# Autodesk Inventor assembly: bunny bot 2013 idea 2.2
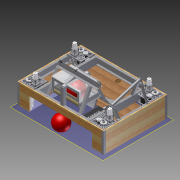
[picture p0: Inventor's stored thumbnail of the model, 180x180]
Saved by Autodesk Inventor 2012 (Build 160160000, 160)
## iProperties
Created: 2013-09-01
Part Number: bunny bot 2013 idea 2.2
Document SubType Name: Assembly
Designer: Bryce
Author: Bryce
## Documents named in this file (30)
- C:\Users\Bryce\Dropbox\Inventor Design Project Files\Independent Swerves\Inventor 2012\bunny bot 2013 idea 2.2.iam
- C:\Users\Bryce\Dropbox\Inventor Design Project Files\Independent Swerves\Inventor 2012\FULL SWERVE DRIVE ASSEMBLY!  2!.iam
- C:\Users\Bryce\Dropbox\Inventor Design Project Files\Independent Swerves\Inventor 2012\frame U 1 by 3.ipt
- C:\Users\Bryce\Dropbox\Inventor Design Project Files\Independent Swerves\Inventor 2012\frame U 1 by 3 long.ipt
- C:\Users\Bryce\Dropbox\Inventor Design Project Files\Independent Swerves\Inventor 2012\plywood side pannel.ipt
- C:\Users\Bryce\Dropbox\Inventor Design Project Files\Independent Swerves\Inventor 2012\plywood back pannel 2.ipt
- C:\Users\Bryce\Dropbox\Inventor Design Project Files\Independent Swerves\Inventor 2012\dozer side pannel.ipt
- C:\Users\Bryce\Dropbox\Inventor Design Project Files\Independent Swerves\Inventor 2012\plywood front pannel 2.ipt
- C:\Users\Bryce\Dropbox\Inventor Design Project Files\Independent Swerves\Inventor 2012\dodge ball.ipt
- C:\Users\Bryce\Dropbox\Inventor Design Project Files\Independent Swerves\Inventor 2012\dozer side end mount.ipt
- C:\Users\Bryce\Dropbox\Inventor Design Project Files\Independent Swerves\Inventor 2012\bumper corner bracket.ipt
- C:\Users\Bryce\Dropbox\Inventor Design Project Files\Independent Swerves\Inventor 2012\dozer side mid mount.ipt
- C:\Users\Bryce\Dropbox\Inventor Design Project Files\Independent Swerves\Inventor 2012\frame box 1 by 3.ipt
- C:\Users\Bryce\Dropbox\Inventor Design Project Files\Independent Swerves\Inventor 2012\belly pan.ipt
- C:\Users\Bryce\Dropbox\Inventor Design Project Files\Independent Swerves\Inventor 2012\8 ball frame tube.ipt
- C:\Users\Bryce\Dropbox\Inventor Design Project Files\Independent Swerves\Inventor 2012\manipulator pnumaitic pivot.ipt
- C:\Users\Bryce\Dropbox\Inventor Design Project Files\Independent Swerves\Inventor 2012\bunny throw base 1.ipt
- C:\Users\Bryce\Dropbox\Inventor Design Project Files\Independent Swerves\Inventor 2012\bunny throw base 2.ipt
- C:\Users\Bryce\Dropbox\Inventor Design Project Files\Independent Swerves\Inventor 2012\1' by 1'' dia piston.ipt
- C:\Users\Bryce\Dropbox\Inventor Design Project Files\Independent Swerves\Inventor 2012\bunny throw piston bracket.ipt
- C:\Users\Bryce\Dropbox\Inventor Design Project Files\Independent Swerves\Inventor 2012\frame U 1 by 3 long 2.ipt
- C:\Users\Bryce\Dropbox\Inventor Design Project Files\Independent Swerves\Inventor 2012\8 ball slider U.ipt
- C:\Users\Bryce\Dropbox\Inventor Design Project Files\Independent Swerves\Inventor 2012\8 ball mechanism 3.iam
- C:\Users\Bryce\Dropbox\Inventor Design Project Files\Independent Swerves\Inventor 2012\8 ball top roller L frame.ipt
- C:\Users\Bryce\Dropbox\Inventor Design Project Files\Independent Swerves\Inventor 2012\8 ball lift frame.ipt
- C:\Users\Bryce\Dropbox\Inventor Design Project Files\Independent Swerves\Inventor 2012\8 ball top roller L frame_MIR.ipt
- C:\Users\Bryce\Dropbox\Inventor Design Project Files\Independent Swerves\Inventor 2012\6''  by 1'' dia piston.ipt
- C:\Users\Bryce\Dropbox\Inventor Design Project Files\Inventor library\Electrical\CRIO Controller\cRIO-FRC.iam
- C:\Users\Bryce\Dropbox\Inventor Design Project Files\Independent Swerves\Inventor 2012\8 ball frame gusset.ipt
- C:\Users\Bryce\Dropbox\Inventor Design Project Files\Independent Swerves\Inventor 2012\8 ball cable roller assembly.iam
## Components (51 placed, 29 different names)
1. FULL SWERVE DRIVE ASSEMBLY!  2!:1 [sub-assembly] — Mate:6, Mate:7, Mate:8
2. FULL SWERVE DRIVE ASSEMBLY!  2!:2 [sub-assembly] — Mate:12, Mate:13, Mate:14
3. FULL SWERVE DRIVE ASSEMBLY!  2!:3 [sub-assembly] — Mate:9, Mate:10, Mate:11
4. FULL SWERVE DRIVE ASSEMBLY!  2!:4 [sub-assembly] — Mate:15, Mate:16, Mate:17, Tangent:1
5. frame U 1 by 3:1 — Mate:1, Mate:2, Flush:1, Mate:5, Mate:14, Mate:15, Mate:35, Flush:8, Flush:26, Flush:27, Flush:51
6. frame U 1 by 3:2 — Mate:3, Mate:4, Flush:2, Flush:3, Mate:6, Mate:7, Mate:9, Mate:10, Mate:34, Flush:6, Flush:25, Flush:28
7. frame U 1 by 3 long:1 — Mate:1, Mate:4, Flush:3, Mate:5, Mate:11, Mate:12, Mate:13, Mate:36, Flush:12, Mate:72, Mate:73, Flush:35, Flush:36, Flush:37, Flush:38
8. frame U 1 by 3 long 2:1 — Mate:2, Mate:3, Flush:1, Flush:2, Mate:8, Mate:16, Mate:17, Flush:7, Flush:9, Flush:13, Mate:46, Mate:103, Mate:104, Flush:52, Mate:128, Mate:133, Mate:143
9. plywood side pannel:1 — Mate:34, Flush:6, Flush:7, Mate:43, Flush:14, Mate:60, Mate:66, Flush:24, Mate:70, Mate:71, Mate:75
10. plywood side pannel:2 — Mate:35, Flush:8, Flush:9, Mate:37, Mate:45, Mate:62, Mate:67, Flush:23, Mate:68, Mate:69, Flush:142
11. plywood back pannel 2:1 — Mate:36, Flush:12, Mate:37, Mate:38, Mate:39, Angle:1, Mate:48, Mate:49, Mate:50, Mate:51, Flush:15, Flush:16, Flush:17, Flush:18, Flush:21, Flush:22, Flush:30, Flush:31, Mate:74
12. dozer side pannel:1 — Mate:38, Mate:43, Mate:53, Mate:55, Mate:56, Flush:29, Flush:30, Flush:32
13. dozer side pannel:2 — Mate:39, Mate:45, Mate:52, Mate:54, Mate:57, Flush:31, Flush:33, Flush:34
14. plywood front pannel 2:2 — Flush:13, Mate:46, Flush:14, Mate:58, Mate:59, Flush:19, Flush:20, Mate:61, Mate:63, Mate:64, Mate:65
15. dozer side end mount:1 — Mate:50, Mate:55, Flush:17
16. dozer side end mount:2 — Mate:48, Mate:53, Flush:18
17. dozer side end mount:3 — Mate:49, Mate:52, Flush:16
18. dozer side end mount:4 — Mate:51, Mate:54, Flush:15
19. dozer side end mount:5 — Mate:56, Mate:59, Flush:19
20. dozer side end mount:6 — Mate:57, Mate:58, Flush:20
21. bumper corner bracket:1 — Mate:62, Mate:67, Flush:22
22. bumper corner bracket:2 — Mate:60, Mate:66, Flush:21
23. bumper corner bracket:3 — Mate:61, Mate:65, Flush:24
24. bumper corner bracket:4 — Mate:63, Mate:64, Flush:23
25. dozer side mid mount:1 — Mate:71, Flush:25, Flush:29
26. dozer side mid mount:2 — Mate:70, Flush:28, Flush:32
27. dozer side mid mount:3 — Mate:68, Flush:27, Flush:34
28. dozer side mid mount:4 — Mate:69, Flush:26, Flush:33
29. frame box 1 by 3:1 — Mate:73, Flush:37, Flush:38, Mate:76, Mate:78, Flush:40, Mate:144, Flush:138
30. frame box 1 by 3:2 — Mate:72, Flush:35, Flush:36, Flush:47, Mate:92, Flush:48, Mate:93, Mate:142, Mate:145, Flush:139
31. belly pan:1 — Mate:74, Mate:75, Mate:76, Mate:141, Mate:146
32. 8 ball frame tube:2 — Mate:78, Flush:40, Mate:107, Flush:53, Flush:129, Flush:134, Flush:140, Flush:141
33. dodge ball:2 — Mate:102
34. bunny throw base 1:1 — Flush:47, Mate:92, Mate:94, Flush:49, Mate:95, Mate:96, Flush:51
35. bunny throw base 2:1 — Flush:48, Mate:93, Mate:94, Flush:50, Mate:99, Mate:100
36. 1' by 1'' dia piston:1 — Mate:97, Mate:98, Mate:101
37. manipulator pnumaitic pivot:2 — Flush:49, Mate:95, Mate:96, Mate:97, Mate:98
38. bunny throw piston bracket:1 — Flush:50, Mate:99, Mate:100, Mate:101
39. 8 ball slider U:1 — Mate:103, Mate:104, Flush:52, Mate:105, Mate:106, Mate:135
40. 8 ball mechanism 3:1 [sub-assembly] — Mate:105, Mate:106, Mate:108, Mate:109, Mate:146
41. 8 ball slider U:2 — Mate:107, Flush:53, Mate:108, Mate:109
42. 8 ball top roller L frame:2 — Mate:130, Mate:131, Flush:135, Mate:139, Flush:137
43. 8 ball lift frame:1 — Mate:133, Flush:134, Mate:135, Flush:137
44. 8 ball lift frame:2 — Mate:128, Flush:129, Mate:130, Mate:131, Mate:140, Flush:142
45. 8 ball top roller L frame_MIR:1 — Mate:136, Mate:137, Mate:138, Mate:139, Mate:140, Angle:2, Mate:147, Mate:148, Mate:149, Mate:150
46. 6''  by 1'' dia piston:1 — Mate:137, Mate:138, Angle:2
47. cRIO-FRC:1 [sub-assembly] — Mate:141, Mate:142, Mate:143
48. 8 ball frame gusset:1 — Mate:144, Flush:138, Flush:141
49. 8 ball frame gusset:2 — Mate:145, Flush:139, Flush:140
50. 8 ball cable roller assembly:1 [sub-assembly] — Mate:147, Mate:149
51. 8 ball cable roller assembly:2 [sub-assembly] — Mate:148, Mate:150
## Relationships (148: Mate 94, Flush 51, Angle 2, Tangent 1)
- Mate:1: frame U 1 by 3:1 ↔ frame U 1 by 3 long:1
- Mate:2: frame U 1 by 3:1 ↔ frame U 1 by 3 long 2:1
- Mate:3: frame U 1 by 3:2 ↔ frame U 1 by 3 long 2:1
- Mate:4: frame U 1 by 3:2 ↔ frame U 1 by 3 long:1
- Flush:1: frame U 1 by 3:1 ↔ frame U 1 by 3 long 2:1
- Flush:2: frame U 1 by 3:2 ↔ frame U 1 by 3 long 2:1
- Flush:3: frame U 1 by 3:2 ↔ frame U 1 by 3 long:1
- Mate:5: frame U 1 by 3:1 ↔ frame U 1 by 3 long:1
- Mate:6: FULL SWERVE DRIVE ASSEMBLY!  2!:1 ↔ frame U 1 by 3:2
- Mate:7: FULL SWERVE DRIVE ASSEMBLY!  2!:1 ↔ frame U 1 by 3:2
- Mate:8: FULL SWERVE DRIVE ASSEMBLY!  2!:1 ↔ frame U 1 by 3 long 2:1
- Mate:9: FULL SWERVE DRIVE ASSEMBLY!  2!:3 ↔ frame U 1 by 3:2
- Mate:10: FULL SWERVE DRIVE ASSEMBLY!  2!:3 ↔ frame U 1 by 3:2
- Mate:11: FULL SWERVE DRIVE ASSEMBLY!  2!:3 ↔ frame U 1 by 3 long:1
- Mate:12: FULL SWERVE DRIVE ASSEMBLY!  2!:2 ↔ frame U 1 by 3 long:1
- Mate:13: FULL SWERVE DRIVE ASSEMBLY!  2!:2 ↔ frame U 1 by 3 long:1
- Mate:14: FULL SWERVE DRIVE ASSEMBLY!  2!:2 ↔ frame U 1 by 3:1
- Mate:15: FULL SWERVE DRIVE ASSEMBLY!  2!:4 ↔ frame U 1 by 3:1
- Mate:16: FULL SWERVE DRIVE ASSEMBLY!  2!:4 ↔ frame U 1 by 3 long 2:1
- Mate:17: FULL SWERVE DRIVE ASSEMBLY!  2!:4 ↔ frame U 1 by 3 long 2:1
- Mate:34: frame U 1 by 3:2 ↔ plywood side pannel:1
- Flush:6: frame U 1 by 3:2 ↔ plywood side pannel:1
- Flush:7: frame U 1 by 3 long 2:1 ↔ plywood side pannel:1
- Mate:35: frame U 1 by 3:1 ↔ plywood side pannel:2
- Flush:8: frame U 1 by 3:1 ↔ plywood side pannel:2
- Flush:9: frame U 1 by 3 long 2:1 ↔ plywood side pannel:2
- Mate:36: frame U 1 by 3 long:1 ↔ plywood back pannel 2:1
- Flush:12: frame U 1 by 3 long:1 ↔ plywood back pannel 2:1
- Mate:37: plywood side pannel:2 ↔ plywood back pannel 2:1
- Mate:38: plywood back pannel 2:1 ↔ dozer side pannel:1
- Mate:39: plywood back pannel 2:1 ↔ dozer side pannel:2
- Mate:43 (114.3 mm): plywood side pannel:1 ↔ dozer side pannel:1
- Mate:45 (114.3 mm): plywood side pannel:2 ↔ dozer side pannel:2
- Flush:13: frame U 1 by 3 long 2:1 ↔ plywood front pannel 2:2
- Mate:46: frame U 1 by 3 long 2:1 ↔ plywood front pannel 2:2
- Flush:14: plywood side pannel:1 ↔ plywood front pannel 2:2
- Angle:1 (0 deg): plywood back pannel 2:1
- Tangent:1: FULL SWERVE DRIVE ASSEMBLY!  2!:4
- Mate:48: plywood back pannel 2:1 ↔ dozer side end mount:2
- Mate:49: plywood back pannel 2:1 ↔ dozer side end mount:3
- Mate:50: plywood back pannel 2:1 ↔ dozer side end mount:1
- Mate:51: plywood back pannel 2:1 ↔ dozer side end mount:4
- Mate:52: dozer side pannel:2 ↔ dozer side end mount:3
- Mate:53: dozer side pannel:1 ↔ dozer side end mount:2
- Mate:54: dozer side pannel:2 ↔ dozer side end mount:4
- Flush:15: plywood back pannel 2:1 ↔ dozer side end mount:4
- Flush:16: plywood back pannel 2:1 ↔ dozer side end mount:3
- Mate:55: dozer side pannel:1 ↔ dozer side end mount:1
- Flush:17: plywood back pannel 2:1 ↔ dozer side end mount:1
- Flush:18: plywood back pannel 2:1 ↔ dozer side end mount:2
- Mate:56: dozer side pannel:1 ↔ dozer side end mount:5
- Mate:57: dozer side pannel:2 ↔ dozer side end mount:6
- Mate:58: plywood front pannel 2:2 ↔ dozer side end mount:6
- Mate:59: plywood front pannel 2:2 ↔ dozer side end mount:5
- Flush:19: plywood front pannel 2:2 ↔ dozer side end mount:5
- Flush:20: plywood front pannel 2:2 ↔ dozer side end mount:6
- Mate:60: plywood side pannel:1 ↔ bumper corner bracket:2
- Mate:61: plywood front pannel 2:2 ↔ bumper corner bracket:3
- Mate:62: plywood side pannel:2 ↔ bumper corner bracket:1
- Mate:63: plywood front pannel 2:2 ↔ bumper corner bracket:4
- Mate:64: plywood front pannel 2:2 ↔ bumper corner bracket:4
- Mate:65: plywood front pannel 2:2 ↔ bumper corner bracket:3
- Mate:66: plywood side pannel:1 ↔ bumper corner bracket:2
- Mate:67: plywood side pannel:2 ↔ bumper corner bracket:1
- Flush:21: plywood back pannel 2:1 ↔ bumper corner bracket:2
- Flush:22: plywood back pannel 2:1 ↔ bumper corner bracket:1
- Flush:23: plywood side pannel:2 ↔ bumper corner bracket:4
- Flush:24: plywood side pannel:1 ↔ bumper corner bracket:3
- Mate:68: plywood side pannel:2 ↔ dozer side mid mount:3
- Mate:69: plywood side pannel:2 ↔ dozer side mid mount:4
- Mate:70: plywood side pannel:1 ↔ dozer side mid mount:2
- Mate:71: plywood side pannel:1 ↔ dozer side mid mount:1
- Flush:25: frame U 1 by 3:2 ↔ dozer side mid mount:1
- Flush:26: frame U 1 by 3:1 ↔ dozer side mid mount:4
- Flush:27: frame U 1 by 3:1 ↔ dozer side mid mount:3
- Flush:28: frame U 1 by 3:2 ↔ dozer side mid mount:2
- Flush:29: dozer side pannel:1 ↔ dozer side mid mount:1
- Flush:30: plywood back pannel 2:1 ↔ dozer side pannel:1
- Flush:31: plywood back pannel 2:1 ↔ dozer side pannel:2
- Flush:32: dozer side pannel:1 ↔ dozer side mid mount:2
- Flush:33: dozer side pannel:2 ↔ dozer side mid mount:4
- Flush:34: dozer side pannel:2 ↔ dozer side mid mount:3
- Mate:72: frame U 1 by 3 long:1 ↔ frame box 1 by 3:2
- Mate:73: frame U 1 by 3 long:1 ↔ frame box 1 by 3:1
- Flush:35: frame U 1 by 3 long:1 ↔ frame box 1 by 3:2
- Flush:36: frame U 1 by 3 long:1 ↔ frame box 1 by 3:2
- Flush:37: frame U 1 by 3 long:1 ↔ frame box 1 by 3:1
- Flush:38: frame U 1 by 3 long:1 ↔ frame box 1 by 3:1
- Mate:74: plywood back pannel 2:1 ↔ belly pan:1
- Mate:75: plywood side pannel:1 ↔ belly pan:1
- Mate:76: frame box 1 by 3:1 ↔ belly pan:1
- Mate:78: frame box 1 by 3:1 ↔ 8 ball frame tube:2
- Flush:40: frame box 1 by 3:1 ↔ 8 ball frame tube:2
- Flush:47: frame box 1 by 3:2 ↔ bunny throw base 1:1
- Mate:92: frame box 1 by 3:2 ↔ bunny throw base 1:1
- Flush:48: frame box 1 by 3:2 ↔ bunny throw base 2:1
- Mate:93: frame box 1 by 3:2 ↔ bunny throw base 2:1
- Mate:94 (298.45 mm): bunny throw base 1:1 ↔ bunny throw base 2:1
- Flush:49: bunny throw base 1:1 ↔ manipulator pnumaitic pivot:2
- Mate:95: bunny throw base 1:1 ↔ manipulator pnumaitic pivot:2
- Mate:96 (-3.175 mm): bunny throw base 1:1 ↔ manipulator pnumaitic pivot:2
- Mate:97: 1' by 1'' dia piston:1 ↔ manipulator pnumaitic pivot:2
- Mate:98 (6.35 mm): 1' by 1'' dia piston:1 ↔ manipulator pnumaitic pivot:2
- Flush:50: bunny throw base 2:1 ↔ bunny throw piston bracket:1
- Mate:99: bunny throw base 2:1 ↔ bunny throw piston bracket:1
- Mate:100 (-1.5875 mm): bunny throw base 2:1 ↔ bunny throw piston bracket:1
- Mate:101: 1' by 1'' dia piston:1 ↔ bunny throw piston bracket:1
- Flush:51: frame U 1 by 3:1 ↔ bunny throw base 1:1
- Mate:102 (-80.01 mm): dodge ball:2
- Mate:103: frame U 1 by 3 long 2:1 ↔ 8 ball slider U:1
- Mate:104: frame U 1 by 3 long 2:1 ↔ 8 ball slider U:1
- Flush:52 (-177.8 mm): frame U 1 by 3 long 2:1 ↔ 8 ball slider U:1
- Mate:105: 8 ball slider U:1 ↔ 8 ball mechanism 3:1
- Mate:106: 8 ball slider U:1 ↔ 8 ball mechanism 3:1
- Mate:107: 8 ball frame tube:2 ↔ 8 ball slider U:2
- Flush:53 (-177.8 mm): 8 ball frame tube:2 ↔ 8 ball slider U:2
- Mate:108: 8 ball mechanism 3:1 ↔ 8 ball slider U:2
- Mate:109: 8 ball mechanism 3:1 ↔ 8 ball slider U:2
- Mate:128: frame U 1 by 3 long 2:1 ↔ 8 ball lift frame:2
- Flush:129: 8 ball frame tube:2 ↔ 8 ball lift frame:2
- Mate:130: 8 ball top roller L frame:2 ↔ 8 ball lift frame:2
- Mate:131: 8 ball top roller L frame:2 ↔ 8 ball lift frame:2
- Mate:133: frame U 1 by 3 long 2:1 ↔ 8 ball lift frame:1
- Flush:134: 8 ball frame tube:2 ↔ 8 ball lift frame:1
- Mate:135 (150.8125 mm): 8 ball slider U:1 ↔ 8 ball lift frame:1
- Flush:135 (9.525 mm): 8 ball top roller L frame:2
- Mate:136 (9.525 mm): 8 ball top roller L frame_MIR:1
- Mate:137: 8 ball top roller L frame_MIR:1 ↔ 6''  by 1'' dia piston:1
- Mate:138 (3.175 mm): 8 ball top roller L frame_MIR:1 ↔ 6''  by 1'' dia piston:1
- Mate:139 (19.05 mm): 8 ball top roller L frame:2 ↔ 8 ball top roller L frame_MIR:1
- Mate:140: 8 ball lift frame:2 ↔ 8 ball top roller L frame_MIR:1
- Flush:137: 8 ball top roller L frame:2 ↔ 8 ball lift frame:1
- Angle:2 (180 deg): 8 ball top roller L frame_MIR:1 ↔ 6''  by 1'' dia piston:1
- Mate:141: belly pan:1 ↔ cRIO-FRC:1
- Mate:142: frame box 1 by 3:2 ↔ cRIO-FRC:1
- Mate:143: frame U 1 by 3 long 2:1 ↔ cRIO-FRC:1
- Mate:144: frame box 1 by 3:1 ↔ 8 ball frame gusset:1
- Mate:145: frame box 1 by 3:2 ↔ 8 ball frame gusset:2
- Flush:138: frame box 1 by 3:1 ↔ 8 ball frame gusset:1
- Flush:139: frame box 1 by 3:2 ↔ 8 ball frame gusset:2
- Flush:140 (-25.4 mm): 8 ball frame tube:2 ↔ 8 ball frame gusset:2
- Flush:141 (-25.4 mm): 8 ball frame tube:2 ↔ 8 ball frame gusset:1
- Mate:146 (12.7 mm): belly pan:1 ↔ 8 ball mechanism 3:1
- Mate:147: 8 ball top roller L frame_MIR:1 ↔ 8 ball cable roller assembly:1
- Mate:148: 8 ball top roller L frame_MIR:1 ↔ 8 ball cable roller assembly:2
- Mate:149 (4.76 mm): 8 ball top roller L frame_MIR:1 ↔ 8 ball cable roller assembly:1
- Mate:150 (4.7625 mm): 8 ball top roller L frame_MIR:1 ↔ 8 ball cable roller assembly:2
- Flush:142 (288.925 mm): plywood side pannel:2 ↔ 8 ball lift frame:2
